# Autodesk Inventor assembly: ABD_RIGHT_OP
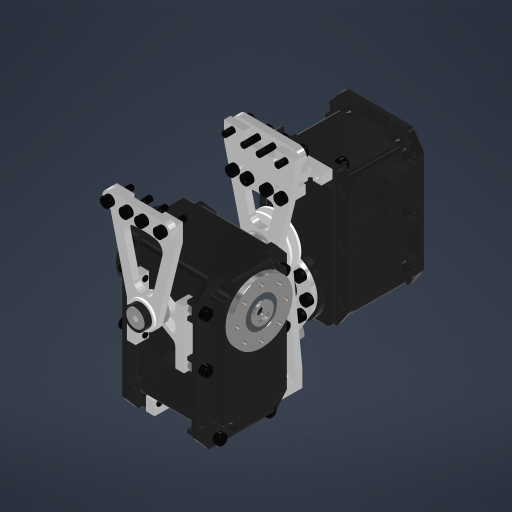
[picture p0: Inventor's stored thumbnail of the model, 512x512]
Saved by Autodesk Inventor 2024 (Build 280153000, 153)
## iProperties
Created: 2024-01-25
Part Number: ABD_RIGHT_OP
Document SubType Name: Assembly
Designer: ASUS
Mass: 367.451 g
Surface Area: 648.88 cm^2
Volume: 184.634 cm^3
Author: ASUS
## Documents named in this file (20)
- C:\Users\ASUS\Desktop\Anti_Backlash_Structure_OP\ABD_RIGHT_OP.iam
- C:\Users\ASUS\Desktop\Anti_Backlash_Structure_OP\MX-106T+idle.ipt.iam
- C:\Users\ASUS\Desktop\Anti_Backlash_Structure_OP\Roll_Fixation_R.ipt
- C:\Users\ASUS\Desktop\Anti_Backlash_Structure_OP\Slider_crank_horn.ipt
- C:\Users\ASUS\Desktop\Anti_Backlash_Structure_OP\Roll_Fixation_L.ipt
- C:\Users\ASUS\Desktop\Anti_Backlash_Structure_OP\Roll_Fixation_Frame.ipt
- C:\Users\ASUS\Desktop\Anti_Backlash_Structure_OP\Leg_joint_slider_frame.ipt
- C:\Users\ASUS\Desktop\Anti_Backlash_Structure_OP\Roll_Fixation_Frame_Back.ipt
- C:\Users\ASUS\Desktop\Anti_Backlash_Structure_OP\106_Slider_Fixation.ipt
- C:\Users\ASUS\Desktop\Anti_Backlash_Structure_OP\hip joint fix washer.ipt
- C:\Users\ASUS\Desktop\Anti_Backlash_Structure_OP\Roll_Fixation_Frameto64.ipt
- C:\Users\ASUS\Desktop\Anti_Backlash_Structure_OP\MISUMI\Roll_Fixation_Frame_8mm_Set.iam
- C:\Users\ASUS\Desktop\Anti_Backlash_Structure_OP\MISUMI\CSH-ST-M2_5-8_203.ipt
- C:\Users\ASUS\Desktop\Anti_Backlash_Structure_OP\MISUMI\hip_joint_fix_washer_10mm_Set.iam
- C:\Users\ASUS\Desktop\Anti_Backlash_Structure_OP\MISUMI\ABD_4mm_set.iam
- C:\Users\ASUS\Desktop\Anti_Backlash_Structure_OP\Front_Frame_Fixer.iam
- C:\Users\ASUS\Desktop\Anti_Backlash_Structure_OP\Rear_Frame_Fixer.iam
- C:\Users\ASUS\Desktop\Anti_Backlash_Structure_OP\Crank_Slider_Fixer.iam
- C:\Users\ASUS\Desktop\Anti_Backlash_Structure_OP\MX-64T.ipt
- MX-106T+idle.ipt
## Components (29 placed, 18 different names)
1. MX-106T+idle.ipt:1 [sub-assembly] — 삽입:8, 메이트:58, 삽입:9, 메이트:59, 삽입:10, 메이트:60
2. Roll_Fixation_R:1 — 메이트:51, 각도:1, 삽입:2
3. Slider_crank_horn:1 — 삽입:3, 삽입:19, 삽입:20, 메이트:69
4. Roll_Fixation_L:1 — 메이트:52, 각도:2, 삽입:4
5. Roll_Fixation_Frame:1 — 메이트:51, 메이트:54
6. Leg_joint_slider_frame:1 — 메이트:53, 삽입:17, 삽입:18, 메이트:63, 메이트:70
7. Roll_Fixation_Frame_Back:1 — 메이트:52, 메이트:53, 플러쉬:1, 삽입:13, 삽입:16, 각도:3
8. 106_Slider_Fixation:1
9. hip joint fix washer:1 — 삽입:5, 메이트:55
10. hip joint fix washer:2 — 삽입:6, 메이트:56
11. Roll_Fixation_Frameto64:1 — 플러쉬:1, 삽입:14, 삽입:15, 메이트:64, 메이트:66, 메이트:68
12. Roll_Fixation_Frame_8mm_Set:1 [sub-assembly] — 삽입:9, 메이트:59
13. Roll_Fixation_Frame_8mm_Set:2 [sub-assembly] — 삽입:10, 메이트:60
14. CSH-ST-M2_5-8_203:1 — 삽입:18
15. CSH-ST-M2_5-8_203:2 — 삽입:17
16. Roll_Fixation_Frame_8mm_Set:3 [sub-assembly] — 삽입:8, 메이트:58
17. hip_joint_fix_washer_10mm_Set:1 [sub-assembly] — 삽입:5, 메이트:55
18. hip_joint_fix_washer_10mm_Set:2 [sub-assembly] — 삽입:6, 메이트:56
19. CSH-ST-M2_5-8_203:3 — 삽입:15
20. CSH-ST-M2_5-8_203:4 — 삽입:13
21. CSH-ST-M2_5-8_203:5 — 삽입:14
22. CSH-ST-M2_5-8_203:6 — 삽입:16
23. Front_Frame_Fixer:1 [sub-assembly] — 각도:1, 삽입:2, 메이트:54
24. Rear_Frame_Fixer:1 [sub-assembly] — 각도:2, 삽입:4
25. Crank_Slider_Fixer:1 [sub-assembly] — 삽입:3, 메이트:63, 메이트:70
26. CSH-ST-M2_5-8_203:7 — 메이트:65, 메이트:66
27. CSH-ST-M2_5-8_203:8 — 메이트:67, 메이트:68
28. MX-64T:1 — 삽입:19, 메이트:64, 메이트:65, 메이트:67
29. ABD_4mm_set:1 [sub-assembly] — 삽입:20, 메이트:69
## Relationships (60: Mate 40, Insert 16, Angle 3, Flush 1)
- [Mate] (0.05 mm): MX-106T+idle.ipt:1 ↔ Roll_Fixation_R:1
- [Mate] (0.05 mm): MX-106T+idle.ipt:1 ↔ Roll_Fixation_L:1
- [Mate]: MX-106T+idle.ipt:1 ↔ Roll_Fixation_L:1
- [Mate]: MX-106T+idle.ipt:1 ↔ Roll_Fixation_L:1
- [Mate]: MX-106T+idle.ipt:1 ↔ Roll_Fixation_L:1
- [Mate]: MX-106T+idle.ipt:1 ↔ Roll_Fixation_R:1
- [Mate]: MX-106T+idle.ipt:1 ↔ Roll_Fixation_R:1
- [Mate]: Roll_Fixation_Frame:1 ↔ Roll_Fixation_Frame_Back:1
- [Mate]: Leg_joint_slider_frame:1 ↔ 106_Slider_Fixation:1
- [Mate]: Leg_joint_slider_frame:1 ↔ 106_Slider_Fixation:1
- [Mate]: Leg_joint_slider_frame:1 ↔ 106_Slider_Fixation:1
- [Mate] (0.05 mm): MX-106T+idle.ipt:1 ↔ 106_Slider_Fixation:1
- [Mate]: MX-106T+idle.ipt:1 ↔ 106_Slider_Fixation:1
- [Mate]: MX-106T+idle.ipt:1 ↔ 106_Slider_Fixation:1
- [Mate]: MX-106T+idle.ipt:1 ↔ 106_Slider_Fixation:1
- [Mate]: Roll_Fixation_Frame:1 ↔ hip joint fix washer:1
- [Mate]: Roll_Fixation_Frame:1 ↔ hip joint fix washer:1
- [Mate]: Roll_Fixation_Frame:1 ↔ hip joint fix washer:1
- [Mate]: Roll_Fixation_Frame_Back:1 ↔ hip joint fix washer:2
- [Mate]: Roll_Fixation_Frame_Back:1 ↔ hip joint fix washer:2
- [Mate]: Roll_Fixation_Frame_Back:1 ↔ hip joint fix washer:2
- [Mate]: Roll_Fixation_Frame_Back:1 ↔ Roll_Fixation_Frameto64:1
- [Mate]: Roll_Fixation_Frame_Back:1 ↔ Roll_Fixation_Frameto64:1
- 메이트:51 [Mate]: Roll_Fixation_R:1 ↔ Roll_Fixation_Frame:1
- 메이트:52 [Mate]: Roll_Fixation_L:1 ↔ Roll_Fixation_Frame_Back:1
- 메이트:53 [Mate]: Leg_joint_slider_frame:1 ↔ Roll_Fixation_Frame_Back:1
- 각도:1 [Angle] (0 deg): Roll_Fixation_R:1 ↔ Front_Frame_Fixer:1
- 삽입:2 [Insert]: Roll_Fixation_R:1 ↔ Front_Frame_Fixer:1
- 삽입:3 [Insert]: Slider_crank_horn:1 ↔ Crank_Slider_Fixer:1
- 각도:2 [Angle] (0 deg): Roll_Fixation_L:1 ↔ Rear_Frame_Fixer:1
- 삽입:4 [Insert]: Roll_Fixation_L:1 ↔ Rear_Frame_Fixer:1
- 메이트:54 [Mate]: Roll_Fixation_Frame:1 ↔ Front_Frame_Fixer:1
- 삽입:5 [Insert]: hip joint fix washer:1 ↔ hip_joint_fix_washer_10mm_Set:1
- 메이트:55 [Mate]: hip joint fix washer:1 ↔ hip_joint_fix_washer_10mm_Set:1
- 삽입:6 [Insert]: hip joint fix washer:2 ↔ hip_joint_fix_washer_10mm_Set:2
- 메이트:56 [Mate]: hip joint fix washer:2 ↔ hip_joint_fix_washer_10mm_Set:2
- 삽입:8 [Insert]: MX-106T+idle.ipt:1 ↔ Roll_Fixation_Frame_8mm_Set:3
- 메이트:58 [Mate]: MX-106T+idle.ipt:1 ↔ Roll_Fixation_Frame_8mm_Set:3
- 삽입:9 [Insert]: MX-106T+idle.ipt:1 ↔ Roll_Fixation_Frame_8mm_Set:1
- 메이트:59 [Mate]: MX-106T+idle.ipt:1 ↔ Roll_Fixation_Frame_8mm_Set:1
- 삽입:10 [Insert]: MX-106T+idle.ipt:1 ↔ Roll_Fixation_Frame_8mm_Set:2
- 메이트:60 [Mate]: MX-106T+idle.ipt:1 ↔ Roll_Fixation_Frame_8mm_Set:2
- 플러쉬:1 [Flush]: Roll_Fixation_Frame_Back:1 ↔ Roll_Fixation_Frameto64:1
- 삽입:13 [Insert]: Roll_Fixation_Frame_Back:1 ↔ CSH-ST-M2_5-8_203:4
- 삽입:14 [Insert]: Roll_Fixation_Frameto64:1 ↔ CSH-ST-M2_5-8_203:5
- 삽입:15 [Insert]: Roll_Fixation_Frameto64:1 ↔ CSH-ST-M2_5-8_203:3
- 삽입:16 [Insert]: Roll_Fixation_Frame_Back:1 ↔ CSH-ST-M2_5-8_203:6
- 삽입:17 [Insert]: Leg_joint_slider_frame:1 ↔ CSH-ST-M2_5-8_203:2
- 삽입:18 [Insert]: Leg_joint_slider_frame:1 ↔ CSH-ST-M2_5-8_203:1
- 삽입:19 [Insert]: Slider_crank_horn:1 ↔ MX-64T:1
- 메이트:63 [Mate]: Leg_joint_slider_frame:1 ↔ Crank_Slider_Fixer:1
- 메이트:64 [Mate]: Roll_Fixation_Frameto64:1 ↔ MX-64T:1
- 메이트:65 [Mate]: CSH-ST-M2_5-8_203:7 ↔ MX-64T:1
- 메이트:66 [Mate]: Roll_Fixation_Frameto64:1 ↔ CSH-ST-M2_5-8_203:7
- 메이트:67 [Mate]: CSH-ST-M2_5-8_203:8 ↔ MX-64T:1
- 메이트:68 [Mate]: Roll_Fixation_Frameto64:1 ↔ CSH-ST-M2_5-8_203:8
- 삽입:20 [Insert]: Slider_crank_horn:1 ↔ ABD_4mm_set:1
- 메이트:69 [Mate]: Slider_crank_horn:1 ↔ ABD_4mm_set:1
- 각도:3 [Angle] (0 deg): Roll_Fixation_Frame_Back:1
- 메이트:70 [Mate] (0.025 mm): Leg_joint_slider_frame:1 ↔ Crank_Slider_Fixer:1
